# Autodesk Inventor assembly: Baugruppe1
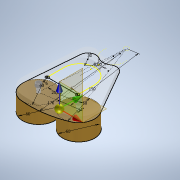
[picture p0: Inventor's stored thumbnail of the model, 180x180]
Saved by Autodesk Inventor 2022 (Build 260153000, 153)
## iProperties
Created: 2022-11-02
Part Number: Baugruppe1
Document SubType Name: Assembly
Designer: alexw
Mass: 1654.54 g
Surface Area: 572.515 cm^2
Volume: 289.304 cm^3
Density: 5.71902 g/cm^3
Author: alexw
## Documents named in this file (6)
- C:\Users\alexw\Documents\Inventor\Projects\03_CurrentProjects\MasterThesis\PSM_V1_Rillenkugellager\Baugruppe1.iam
- C:\Users\alexw\Documents\Inventor\Projects\03_CurrentProjects\MasterThesis\PSM_V1_Rillenkugellager\DPM_Counterweight_Fixation.ipt
- C:\Users\alexw\Documents\Inventor\Projects\03_CurrentProjects\MasterThesis\PSM_V1_Rillenkugellager\DPMAxis1_Weights.ipt
- C:\Users\alexw\Documents\Inventor\Projects\03_CurrentProjects\MasterThesis\PSM_V1_Rillenkugellager\ContentCenter\de-DE\ISO 4762(2)\ISO 4762 - M6 x 50ISO.ipt
- C:\Users\alexw\Documents\Inventor\Projects\03_CurrentProjects\MasterThesis\PSM_V1_Rillenkugellager\ContentCenter\de-DE\ISO 7092\ISO 7092 - ST 6 - 140 HV.ipt
- C:\Users\alexw\Documents\Inventor\Projects\03_CurrentProjects\MasterThesis\PSM_V1_Rillenkugellager\ContentCenter\de-DE\ISO 4032(2)\ISO 4032 - M6 - ISO.ipt
## Components (9 placed, 5 different names)
1. DPM_Counterweight_Fixation:1 — Passend:1, Passend:2, Passend:3, Passend:4, Passend:5, Passend:6, Passend:7, Passend:8
2. DPMAxis1_Weights:1 — Passend:1, Passend:2, Passend:12
3. DPMAxis1_Weights:2 — Passend:3, Passend:4, Passend:10
4. ISO 4762 M6 x 50:1 — Passend:5, Passend:6, Passend:9, Passend:13
5. ISO 4762 M6 x 50:2 — Passend:7, Passend:8, Passend:11, Passend:15
6. ISO 7092 ST 6 - 140 HV:1 — Passend:9, Passend:10, Passend:14
7. ISO 7092 ST 6 - 140 HV:2 — Passend:11, Passend:12, Passend:16
8. ISO 4032 M6:1 — Passend:13, Passend:14
9. ISO 4032 M6:2 — Passend:15, Passend:16
## Relationships (16: Mate 16)
- Passend:1 [Mate]: DPM_Counterweight_Fixation:1 ↔ DPMAxis1_Weights:1
- Passend:2 [Mate]: DPM_Counterweight_Fixation:1 ↔ DPMAxis1_Weights:1
- Passend:3 [Mate]: DPM_Counterweight_Fixation:1 ↔ DPMAxis1_Weights:2
- Passend:4 [Mate]: DPM_Counterweight_Fixation:1 ↔ DPMAxis1_Weights:2
- Passend:5 [Mate]: DPM_Counterweight_Fixation:1 ↔ ISO 4762 M6 x 50:1
- Passend:6 [Mate]: DPM_Counterweight_Fixation:1 ↔ ISO 4762 M6 x 50:1
- Passend:7 [Mate]: DPM_Counterweight_Fixation:1 ↔ ISO 4762 M6 x 50:2
- Passend:8 [Mate]: DPM_Counterweight_Fixation:1 ↔ ISO 4762 M6 x 50:2
- Passend:9 [Mate]: ISO 4762 M6 x 50:1 ↔ ISO 7092 ST 6 - 140 HV:1
- Passend:10 [Mate]: DPMAxis1_Weights:2 ↔ ISO 7092 ST 6 - 140 HV:1
- Passend:11 [Mate]: ISO 4762 M6 x 50:2 ↔ ISO 7092 ST 6 - 140 HV:2
- Passend:12 [Mate]: DPMAxis1_Weights:1 ↔ ISO 7092 ST 6 - 140 HV:2
- Passend:13 [Mate]: ISO 4762 M6 x 50:1 ↔ ISO 4032 M6:1
- Passend:14 [Mate]: ISO 7092 ST 6 - 140 HV:1 ↔ ISO 4032 M6:1
- Passend:15 [Mate]: ISO 4762 M6 x 50:2 ↔ ISO 4032 M6:2
- Passend:16 [Mate]: ISO 7092 ST 6 - 140 HV:2 ↔ ISO 4032 M6:2
